# Autodesk Inventor assembly: main backup 2-6-2020
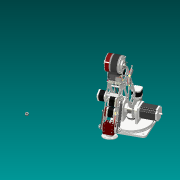
[picture p0: Inventor's stored thumbnail of the model, 180x180]
Saved by Autodesk Inventor 2020 (Build 240168000, 168)
## iProperties
Created: 2020-05-24
Part Number: main backup 2-6-2020
Document SubType Name: Assembly
Designer: Svend
Author: Svend
## Documents named in this file (6)
- D:\github_gedeeld\BeerMinder\3D-model\mainAssembly\main backup 2-6-2020.iam
- D:\github_gedeeld\BeerMinder\3D-model\axis3\axis3.iam
- D:\github_gedeeld\BeerMinder\3D-model\Base (Axis 1)\gefreesd\AssemblyGefreesdBasev2.iam
- D:\github_gedeeld\BeerMinder\3D-model\axis5_6\axis5_6  compact.iam
- D:\github_gedeeld\BeerMinder\3D-model\ControlBox\swithces\Assembly - V-156-1C25 micro switch (Idle).iam
- D:\github_gedeeld\BeerMinder\3D-model\gripper\gripper.iam
## Components (9 placed, 5 different names)
1. axis3:1 [sub-assembly] — Mate:3, Mate:4, Mate:12, Mate:13, Angle:5, Mate:17, Mate:18, Mate:19, Mate:20, Mate:21, Mate:22, Mate:23, Angle:6, Mate:24, Mate:25
2. AssemblyGefreesdBasev2:1 [sub-assembly] — Mate:1, Mate:2, Flush:1, Mate:3, Mate:4, Mate:9, Mate:10, Angle:2, Flush:3
3. axis5_6  compact:1 [sub-assembly] — Mate:12, Mate:13, Mate:14, Mate:15, Angle:5, Angle:6
4. Assembly - V-156-1C25 micro switch (Idle):2 [sub-assembly]
5. Assembly - V-156-1C25 micro switch (Idle):1 [sub-assembly] — Mate:9, Mate:10, Angle:2, Flush:3
6. Assembly - V-156-1C25 micro switch (Idle):3 [sub-assembly] — Mate:20, Mate:21, Mate:22
7. gripper:1 [sub-assembly] — Mate:14, Mate:15
8. Assembly - V-156-1C25 micro switch (Idle):4 [sub-assembly] — Mate:17, Mate:18, Mate:19
9. Assembly - V-156-1C25 micro switch (Idle):5 [sub-assembly] — Mate:23, Mate:24, Mate:25
## Relationships (27: Mate 20, Angle 4, Flush 3)
- Mate:1: AssemblyGefreesdBasev2:1
- Mate:2: AssemblyGefreesdBasev2:1
- Flush:1: AssemblyGefreesdBasev2:1
- Mate:3: axis3:1 ↔ AssemblyGefreesdBasev2:1
- Mate:4: axis3:1 ↔ AssemblyGefreesdBasev2:1
- [Mate] (2 mm): AssemblyGefreesdBasev2:1 ↔ Assembly - V-156-1C25 micro switch (Idle):2
- [Angle] (180 deg): AssemblyGefreesdBasev2:1 ↔ Assembly - V-156-1C25 micro switch (Idle):2
- [Flush] (19 mm): AssemblyGefreesdBasev2:1 ↔ Assembly - V-156-1C25 micro switch (Idle):2
- Mate:9 (95 mm): AssemblyGefreesdBasev2:1 ↔ Assembly - V-156-1C25 micro switch (Idle):1
- Mate:10: AssemblyGefreesdBasev2:1 ↔ Assembly - V-156-1C25 micro switch (Idle):1
- Angle:2 (0 deg): AssemblyGefreesdBasev2:1 ↔ Assembly - V-156-1C25 micro switch (Idle):1
- Flush:3 (35 mm): AssemblyGefreesdBasev2:1 ↔ Assembly - V-156-1C25 micro switch (Idle):1
- Mate:12: axis3:1 ↔ axis5_6  compact:1
- Mate:13: axis3:1 ↔ axis5_6  compact:1
- Mate:14: axis5_6  compact:1 ↔ gripper:1
- Mate:15: axis5_6  compact:1 ↔ gripper:1
- Angle:5 (310 deg): axis3:1 ↔ axis5_6  compact:1
- Mate:17: axis3:1 ↔ Assembly - V-156-1C25 micro switch (Idle):4
- Mate:18: axis3:1 ↔ Assembly - V-156-1C25 micro switch (Idle):4
- Mate:19: axis3:1 ↔ Assembly - V-156-1C25 micro switch (Idle):4
- Mate:20: axis3:1 ↔ Assembly - V-156-1C25 micro switch (Idle):3
- Mate:21: axis3:1 ↔ Assembly - V-156-1C25 micro switch (Idle):3
- Mate:22: axis3:1 ↔ Assembly - V-156-1C25 micro switch (Idle):3
- Mate:23: axis3:1 ↔ Assembly - V-156-1C25 micro switch (Idle):5
- Angle:6 (0 deg): axis3:1 ↔ axis5_6  compact:1
- Mate:24: axis3:1 ↔ Assembly - V-156-1C25 micro switch (Idle):5
- Mate:25: axis3:1 ↔ Assembly - V-156-1C25 micro switch (Idle):5
